# Autodesk Inventor assembly: 2 x AA Battery Holder
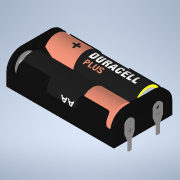
[picture p0: Inventor's stored thumbnail of the model, 180x180]
Saved by Autodesk Inventor 2020 (Build 240168000, 168)
## iProperties
Created: 2021-12-31
Part Number: 2 x AA Battery Holder
Document SubType Name: Assembly
Designer: robur
Author: robur
## iProperties of the stored document AA Duracell Body.ipt
Created: 2011-12-10
Part Number: AA Duracell Body
Material: Generic
Document SubType Name: Modeling
Designer: robur
Density: 1 g/cm^3
Appearance: Default
Sending System: SolidWorks 2011
Last Author: Brads
Last Saved: 2011-12-11
Author: robur
## Documents named in this file (8)
- D:\KiCad Projects\My Libraries\Battery holder\2 x AA Battery Holder .iam
- D:\KiCad Projects\My Libraries\Battery holder\Main body.ipt
- **D:\KiCad Projects\My Libraries\Battery holder\2 x AA Battery Holder .iam*LocalDocs*xAaaaqzcaAaaaaaaaAaaaa1ixPa*AA Duracell Body.ipt
- D:\KiCad Projects\My Libraries\Battery holder\Spring.ipt
- D:\KiCad Projects\My Libraries\Battery holder\Contact.ipt
- D:\KiCad Projects\My Libraries\Battery holder\Positive Pin.ipt
- D:\KiCad Projects\My Libraries\Battery holder\Negative Pin.ipt
- D:\KiCad Projects\My Libraries\Battery holder\AA Duracell Body.SLDPRT
## Components (9 placed, 6 different names)
1. Main body:1 — Insert:1, Insert:4, Mate:1, Insert:5, Insert:9
2. AA Duracell Body:1 — Insert:7
3. AA Duracell Body:2 — Insert:2
4. Spring:2 — Insert:5
5. Spring:3 — Insert:4
6. Contact:1 — Mate:1, Insert:7
7. Contact:2 — Insert:1, Insert:2, Insert:8
8. Positive Pin:2 — Insert:8
9. Negative Pin:2 — Insert:9
## Relationships (8: Insert 7, Mate 1)
- Insert:1: Main body:1 ↔ Contact:2
- Insert:2: AA Duracell Body:2 ↔ Contact:2
- Insert:4: Main body:1 ↔ Spring:3
- Mate:1: Main body:1 ↔ Contact:1
- Insert:5: Main body:1 ↔ Spring:2
- Insert:7: AA Duracell Body:1 ↔ Contact:1
- Insert:8: Contact:2 ↔ Positive Pin:2
- Insert:9: Main body:1 ↔ Negative Pin:2
